# Autodesk Inventor assembly: 276-2154
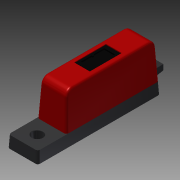
[picture p0: Inventor's stored thumbnail of the model, 180x180]
Saved by Autodesk Inventor 2015 (Build 190159000, 159)
## iProperties
Company: Bots 'n' Stuff
Created: 2011-10-10
Part Number: 276-2154
Catalog Web Link: http://vexrobotics.com/276-2154.html
Vendor: VEX Robotics, Inc.
Document SubType Name: Assembly
Designer: Jordan Kiesel
Mass: 15.4227 g
Surface Area: 87.666 cm^2
Volume: 6.02022 cm^3
Density: 2.56181 g/cm^3
Title: Line Tracker
Author: Jordan Kiesel
## Documents named in this file (6)
- C:\Users\Jordan\Documents\Robotics\CAD\2015 BNS CAD Library (beta)\Sensors\Line Tracker.iam
- C:\Users\Jordan\Documents\Robotics\CAD\2015 BNS CAD Library (beta)\Sensors\Reference Parts\Line Tracker\Sensor Module Top.ipt
- C:\Users\Jordan\Documents\Robotics\CAD\2015 BNS CAD Library (beta)\Sensors\Reference Parts\Line Tracker\PCB.ipt
- C:\Users\Jordan\Documents\Robotics\CAD\2015 BNS CAD Library (beta)\Sensors\Reference Parts\Line Tracker\Sensor Module Bottom.ipt
- C:\Users\Jordan\Documents\Robotics\CAD\2015 BNS CAD Library (beta)\Sensors\Reference Parts\Line Tracker\Set Screw M2x8.ipt
- C:\Users\Jordan\Documents\Robotics\CAD\2015 BNS CAD Library (beta)\Sensors\Reference Parts\Line Tracker\Grommet.ipt
## Components (6 placed, 5 different names)
1. Sensor Module Bottom:1 — Insert:1, Insert:2, Insert:3, Insert:4, Mate:2, Mate:3
2. PCB:1 — Insert:1, Insert:2, Insert:5, Insert:6
3. Set Screw M2x8:1 — Insert:3
4. Set Screw M2x8:2 — Insert:4
5. Sensor Module Top:1 — Insert:5, Insert:6, Mate:1
6. Grommet:1 — Mate:1, Mate:2, Mate:3
## Relationships (9: Insert 6, Mate 3)
- Insert:1: Sensor Module Bottom:1 ↔ PCB:1
- Insert:2: Sensor Module Bottom:1 ↔ PCB:1
- Insert:3: Sensor Module Bottom:1 ↔ Set Screw M2x8:1
- Insert:4: Sensor Module Bottom:1 ↔ Set Screw M2x8:2
- Mate:1: Sensor Module Top:1 ↔ Grommet:1
- Mate:2: Sensor Module Bottom:1 ↔ Grommet:1
- Mate:3: Sensor Module Bottom:1 ↔ Grommet:1
- Insert:5: PCB:1 ↔ Sensor Module Top:1
- Insert:6: PCB:1 ↔ Sensor Module Top:1
